# Autodesk Inventor assembly: s-assy-shooter_unit
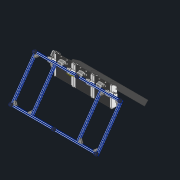
[picture p0: Inventor's stored thumbnail of the model, 180x180]
Saved by Autodesk Inventor 2022 (Build 260153000, 153)
## iProperties
Created: 2021-08-20
Part Number: s-assy-shooter_unit
Document SubType Name: Assembly
Designer: yuta0
Mass: 2841.37 g
Surface Area: 10239.2 cm^2
Volume: 1741.74 cm^3
Density: 1.63133 g/cm^3
Author: yuta0
## Documents named in this file (20)
- C:\Users\yuta0\Documents\GitHub\catchrobo_hardware\assy-shooter\assy-shooter.iam
- C:\Users\yuta0\Documents\GitHub\catchrobo_hardware\assy-shooter\shooter_carbon_plate1.ipt
- C:\Users\yuta0\Documents\GitHub\catchrobo_hardware\assy-shooter\shooter_base4.ipt
- C:\Users\yuta0\Documents\GitHub\catchrobo_hardware\assy-shooter\MF126ZZ.ipt
- C:\Users\yuta0\Documents\GitHub\catchrobo_hardware\assy-shooter\s-assy-sorter_motor.iam
- C:\Users\yuta0\Documents\GitHub\catchrobo_hardware\assy-shooter\s-assy-shooter_motor2.iam
- C:\Users\yuta0\Documents\GitHub\catchrobo_hardware\assy-shooter\s-assy-sorter_plate.iam
- C:\Users\yuta0\Documents\GitHub\catchrobo_hardware\assy-shooter\s-assy-guide_plates.iam
- C:\Users\yuta0\Documents\GitHub\catchrobo_hardware\assy-shooter\CBSTSR3-10.ipt
- C:\Users\yuta0\Documents\GitHub\catchrobo_hardware\assy-shooter\LBNR3.ipt
- C:\Users\yuta0\Documents\GitHub\catchrobo_hardware\assy-shooter\CB3-15.ipt
- C:\Users\yuta0\Documents\GitHub\catchrobo_hardware\assy-shooter\shooter_base1.ipt
- C:\Users\yuta0\Documents\GitHub\catchrobo_hardware\assy-shooter\s-assy-frame-connector.iam
- C:\Users\yuta0\Documents\GitHub\catchrobo_hardware\assy-shooter\s-assy-shooter_frame.iam
- C:\Users\yuta0\Documents\GitHub\catchrobo_hardware\assy-shooter\s-assy-bearing_stopper.iam
- C:\Users\yuta0\Documents\GitHub\catchrobo_hardware\assy-shooter\d_type_board.ipt
- C:\Users\yuta0\Documents\GitHub\catchrobo_hardware\assy-shooter\hexagonal_spacer_M3_5mm.ipt
- C:\Users\yuta0\Documents\GitHub\catchrobo_hardware\assy-shooter\CB3-5.ipt
- C:\Users\yuta0\Documents\GitHub\catchrobo_hardware\assy-shooter\shooter_base8[.ipt
- C:\Users\yuta0\Documents\GitHub\catchrobo_hardware\assy-shooter\Part2.ipt
## Components (97 placed, 19 different names)
1. s-assy-shooter_motor2:1 [sub-assembly] — メイト:215, メイト:222, メイト:280, メイト:282, メイト:283, メイト:307, メイト:308, メイト:309
2. s-assy-guide_plates:1 [sub-assembly] — メイト:222, 角度:2, メイト:280, メイト:285, メイト:293, メイト:302
3. s-assy-shooter_frame:1 [sub-assembly] — メイト:272, メイト:273, フラッシュ:10
4. s-assy-bearing_stopper:7 [sub-assembly] — メイト:279, メイト:301, メイト:302
5. MF126ZZ:2 — メイト:56, メイト:281
6. MF126ZZ:9 — メイト:279, メイト:301, メイト:303
7. d_type_board:1 — メイト:294, メイト:295, メイト:298, メイト:299, メイト:300
8. shooter_base8[:1 — メイト:304, メイト:305, メイト:306
9. shooter_base8[:2 — メイト:307, メイト:308, メイト:309, フラッシュ:11, メイト:310
10. Part2:1 — フラッシュ:11, メイト:310
11. s-assy-frame-connector:3 [sub-assembly] — メイト:271, メイト:272, メイト:273, メイト:292
12. s-assy-frame-connector:4 [sub-assembly] — メイト:294, メイト:295, メイト:296, メイト:297
13. s-assy-frame-connector:5 [sub-assembly]
14. s-assy-frame-connector:6 [sub-assembly]
15. shooter_carbon_plate1:1 — メイト:20, メイト:21, フラッシュ:6, メイト:209, メイト:210, メイト:212, メイト:223, メイト:224, メイト:250, メイト:284, メイト:286, メイト:287
16. shooter_base4:1 — メイト:20, メイト:21, フラッシュ:6, メイト:53, メイト:54, メイト:56, メイト:215, メイト:226, メイト:271, フラッシュ:10, メイト:281, メイト:282, メイト:283
17. shooter_base1:1 — メイト:248, メイト:249, メイト:250, メイト:252, 角度:3, メイト:256, メイト:257, メイト:258, メイト:260, メイト:261, メイト:284
18. s-assy-sorter_plate:1 [sub-assembly] — メイト:217, メイト:218, 角度:1
19. s-assy-sorter_motor:1 [sub-assembly] — メイト:209, メイト:210, メイト:212, メイト:217, メイト:218, 角度:1
20. s-assy-bearing_stopper:2 [sub-assembly] — メイト:277, メイト:293
21. MF126ZZ:4 — メイト:252, メイト:277, メイト:285
22. s-assy-bearing_stopper:1 [sub-assembly] — メイト:275
23. MF126ZZ:1 — メイト:53, メイト:54, メイト:275
24. shooter_carbon_plate1:2
25. shooter_base4:2 — メイト:288, メイト:289, メイト:290, メイト:291
26. shooter_base1:2
27. s-assy-sorter_plate:2 [sub-assembly]
28. s-assy-sorter_motor:2 [sub-assembly]
29. s-assy-bearing_stopper:8 [sub-assembly]
30. MF126ZZ:10
31. s-assy-bearing_stopper:10 [sub-assembly]
32. MF126ZZ:12
33. shooter_carbon_plate1:3
34. shooter_base4:3
35. shooter_base1:3 — メイト:303, メイト:304, メイト:305, メイト:306
36. s-assy-sorter_plate:3 [sub-assembly]
37. s-assy-sorter_motor:3 [sub-assembly]
38. s-assy-bearing_stopper:9 [sub-assembly]
39. MF126ZZ:11
40. s-assy-bearing_stopper:11 [sub-assembly]
41. MF126ZZ:13
42. LBNR3:18 — メイト:247, 角度:3, 角度:4, フラッシュ:9
43. LBNR3:17 — メイト:245, 角度:4, 角度:5, フラッシュ:8, フラッシュ:9
44. LBNR3:16 — メイト:243, 角度:6, フラッシュ:7, フラッシュ:8, メイト:256
45. LBNR3:15 — メイト:241, 角度:5, 角度:6, フラッシュ:7
46. CB3-15:4 — メイト:241, メイト:257, メイト:289
47. CB3-15:3 — メイト:243, メイト:261, メイト:288
48. CB3-15:2 — メイト:247, メイト:260, メイト:291
49. CB3-15:1 — メイト:245, メイト:258, メイト:290
50. LBNR3:27
51. LBNR3:28
52. LBNR3:29
53. LBNR3:30
54. CB3-15:5
55. CB3-15:6
56. CB3-15:7
57. CB3-15:8
58. hexagonal_spacer_M3_5mm:1 — メイト:296, メイト:297
59. CB3-5:1 — メイト:299, メイト:300
60. hexagonal_spacer_M3_5mm:2 — メイト:298
61. CB3-5:2
62. CBSTSR3-10:1 — メイト:223, メイト:224, メイト:225
63. LBNR3:1 — メイト:225, メイト:226
64. CBSTSR3-10:2
65. LBNR3:2
66. CBSTSR3-10:3 — メイト:248
67. LBNR3:3
68. CBSTSR3-10:4 — メイト:249
69. LBNR3:4
70. CBSTSR3-10:5 — メイト:286, メイト:287, メイト:292
71. CBSTSR3-10:6
72. CBSTSR3-10:7
73. CBSTSR3-10:8
74. CBSTSR3-10:9
75. LBNR3:19
76. CBSTSR3-10:10
77. LBNR3:20
78. CBSTSR3-10:11
79. LBNR3:21
80. CBSTSR3-10:12
81. LBNR3:22
82. CBSTSR3-10:13
83. CBSTSR3-10:14
84. CBSTSR3-10:15
85. CBSTSR3-10:16
86. CBSTSR3-10:17
87. LBNR3:23
88. CBSTSR3-10:18
89. LBNR3:24
90. CBSTSR3-10:19
91. LBNR3:25
92. CBSTSR3-10:20
93. LBNR3:26
94. CBSTSR3-10:21
95. CBSTSR3-10:22
96. CBSTSR3-10:23
97. CBSTSR3-10:24
## Component patterns: (4 elements, first: s-assy-frame-connector:3), (3 elements, first: shooter_carbon_plate1:1 + shooter_base4:1 + shooter_base1:1 + s-assy-sorter_plate:1 + s-assy-sorter_motor:1 + s-assy-bearing_stopper:2 + MF126ZZ:4 + s-assy-bearing_stopper:1 + MF126ZZ:1), (2 elements, first: LBNR3:18 + LBNR3:17 + LBNR3:16 + LBNR3:15 + CB3-15:4 + CB3-15:3 + CB3-15:2 + CB3-15:1), (2 elements, first: hexagonal_spacer_M3_5mm:1 + CB3-5:1), (4 elements, first: CBSTSR3-10:1 + LBNR3:1), (4 elements, first: CBSTSR3-10:5), コンポーネント パターン 4:2 (4 elements), コンポーネント パターン 12:2 (4 elements), コンポーネント パターン 4:3 (4 elements), コンポーネント パターン 12:3 (4 elements)
## Relationships (78: Mate 66, Angle 6, Flush 6)
- 角度:1 [Angle] (0 deg): s-assy-sorter_plate:1 ↔ s-assy-sorter_motor:1
- 角度:2 [Angle] (135 deg): s-assy-guide_plates:1
- メイト:20 [Mate]: shooter_carbon_plate1:1 ↔ shooter_base4:1
- メイト:21 [Mate]: shooter_carbon_plate1:1 ↔ shooter_base4:1
- フラッシュ:6 [Flush]: shooter_carbon_plate1:1 ↔ shooter_base4:1
- メイト:53 [Mate]: shooter_base4:1 ↔ MF126ZZ:1
- メイト:54 [Mate]: shooter_base4:1 ↔ MF126ZZ:1
- メイト:56 [Mate]: MF126ZZ:2 ↔ shooter_base4:1
- メイト:209 [Mate]: shooter_carbon_plate1:1 ↔ s-assy-sorter_motor:1
- メイト:210 [Mate]: shooter_carbon_plate1:1 ↔ s-assy-sorter_motor:1
- メイト:212 [Mate]: shooter_carbon_plate1:1 ↔ s-assy-sorter_motor:1
- メイト:215 [Mate]: s-assy-shooter_motor2:1 ↔ shooter_base4:1
- メイト:217 [Mate]: s-assy-sorter_plate:1 ↔ s-assy-sorter_motor:1
- メイト:218 [Mate]: s-assy-sorter_plate:1 ↔ s-assy-sorter_motor:1
- メイト:222 [Mate]: s-assy-shooter_motor2:1 ↔ s-assy-guide_plates:1
- メイト:223 [Mate]: shooter_carbon_plate1:1 ↔ CBSTSR3-10:1
- メイト:224 [Mate]: shooter_carbon_plate1:1 ↔ CBSTSR3-10:1
- メイト:225 [Mate]: CBSTSR3-10:1 ↔ LBNR3:1
- メイト:226 [Mate]: shooter_base4:1 ↔ LBNR3:1
- メイト:241 [Mate]: LBNR3:15 ↔ CB3-15:4
- メイト:243 [Mate]: LBNR3:16 ↔ CB3-15:3
- メイト:245 [Mate]: LBNR3:17 ↔ CB3-15:1
- メイト:247 [Mate]: LBNR3:18 ↔ CB3-15:2
- メイト:248 [Mate]: shooter_base1:1 ↔ CBSTSR3-10:3
- メイト:249 [Mate]: shooter_base1:1 ↔ CBSTSR3-10:4
- メイト:250 [Mate]: shooter_carbon_plate1:1 ↔ shooter_base1:1
- メイト:252 [Mate]: shooter_base1:1 ↔ MF126ZZ:4
- 角度:3 [Angle] (0 deg): shooter_base1:1 ↔ LBNR3:18
- 角度:4 [Angle] (0 deg): LBNR3:18 ↔ LBNR3:17
- 角度:5 [Angle] (0 deg): LBNR3:17 ↔ LBNR3:15
- 角度:6 [Angle] (0 deg): LBNR3:16 ↔ LBNR3:15
- フラッシュ:7 [Flush]: LBNR3:16 ↔ LBNR3:15
- フラッシュ:8 [Flush]: LBNR3:17 ↔ LBNR3:16
- フラッシュ:9 [Flush]: LBNR3:18 ↔ LBNR3:17
- メイト:256 [Mate]: shooter_base1:1 ↔ LBNR3:16
- メイト:257 [Mate]: shooter_base1:1 ↔ CB3-15:4
- メイト:258 [Mate]: shooter_base1:1 ↔ CB3-15:1
- メイト:260 [Mate]: shooter_base1:1 ↔ CB3-15:2
- メイト:261 [Mate]: shooter_base1:1 ↔ CB3-15:3
- メイト:271 [Mate]: s-assy-frame-connector:3 ↔ shooter_base4:1
- メイト:272 [Mate]: s-assy-shooter_frame:1 ↔ s-assy-frame-connector:3
- メイト:273 [Mate]: s-assy-shooter_frame:1 ↔ s-assy-frame-connector:3
- フラッシュ:10 [Flush] (-150 mm): s-assy-shooter_frame:1 ↔ shooter_base4:1
- メイト:275 [Mate]: s-assy-bearing_stopper:1 ↔ MF126ZZ:1
- メイト:277 [Mate]: s-assy-bearing_stopper:2 ↔ MF126ZZ:4
- メイト:279 [Mate]: s-assy-bearing_stopper:7 ↔ MF126ZZ:9
- メイト:280 [Mate]: s-assy-shooter_motor2:1 ↔ s-assy-guide_plates:1
- メイト:281 [Mate]: MF126ZZ:2 ↔ shooter_base4:1
- メイト:282 [Mate]: s-assy-shooter_motor2:1 ↔ shooter_base4:1
- メイト:283 [Mate]: s-assy-shooter_motor2:1 ↔ shooter_base4:1
- メイト:284 [Mate]: shooter_carbon_plate1:1 ↔ shooter_base1:1
- メイト:285 [Mate]: s-assy-guide_plates:1 ↔ MF126ZZ:4
- メイト:286 [Mate]: shooter_carbon_plate1:1 ↔ CBSTSR3-10:5
- メイト:287 [Mate]: shooter_carbon_plate1:1 ↔ CBSTSR3-10:5
- メイト:288 [Mate]: shooter_base4:2 ↔ CB3-15:3
- メイト:289 [Mate]: shooter_base4:2 ↔ CB3-15:4
- メイト:290 [Mate]: shooter_base4:2 ↔ CB3-15:1
- メイト:291 [Mate]: shooter_base4:2 ↔ CB3-15:2
- メイト:292 [Mate]: s-assy-frame-connector:3 ↔ CBSTSR3-10:5
- メイト:293 [Mate]: s-assy-guide_plates:1 ↔ s-assy-bearing_stopper:2
- メイト:294 [Mate]: d_type_board:1 ↔ s-assy-frame-connector:4
- メイト:295 [Mate]: d_type_board:1 ↔ s-assy-frame-connector:4
- メイト:296 [Mate]: s-assy-frame-connector:4 ↔ hexagonal_spacer_M3_5mm:1
- メイト:297 [Mate]: s-assy-frame-connector:4 ↔ hexagonal_spacer_M3_5mm:1
- メイト:298 [Mate]: d_type_board:1 ↔ hexagonal_spacer_M3_5mm:2
- メイト:299 [Mate]: d_type_board:1 ↔ CB3-5:1
- メイト:300 [Mate]: d_type_board:1 ↔ CB3-5:1
- メイト:301 [Mate]: s-assy-bearing_stopper:7 ↔ MF126ZZ:9
- メイト:302 [Mate]: s-assy-guide_plates:1 ↔ s-assy-bearing_stopper:7
- メイト:303 [Mate]: MF126ZZ:9 ↔ shooter_base1:3
- メイト:304 [Mate]: shooter_base8[:1 ↔ shooter_base1:3
- メイト:305 [Mate]: shooter_base8[:1 ↔ shooter_base1:3
- メイト:306 [Mate]: shooter_base8[:1 ↔ shooter_base1:3
- メイト:307 [Mate]: s-assy-shooter_motor2:1 ↔ shooter_base8[:2
- メイト:308 [Mate]: s-assy-shooter_motor2:1 ↔ shooter_base8[:2
- メイト:309 [Mate]: s-assy-shooter_motor2:1 ↔ shooter_base8[:2
- フラッシュ:11 [Flush]: shooter_base8[:2 ↔ Part2:1
- メイト:310 [Mate]: shooter_base8[:2 ↔ Part2:1
